# Autodesk Inventor assembly: A2017_T5_01
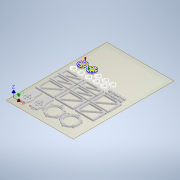
[picture p0: Inventor's stored thumbnail of the model, 180x180]
Saved by Autodesk Inventor 2020 (Build 240168000, 168)
## iProperties
Created: 2021-08-27
Part Number: A2017_T5_01
Document SubType Name: Assembly
Designer: Masato
Author: Masato
## Documents named in this file (9)
- C:\Users\marin\Documents\0113 git clone\OpenPlatform_ver3_0\cam\A2017_T5_01.iam
- C:\Users\marin\Documents\0113 git clone\OpenPlatform_ver3_0\cam\Disposable_Board.ipt
- C:\Users\marin\Documents\0113 git clone\OpenPlatform_ver3_0\LowerBody\Leg_joit\Leg_joint_yaw_frame.ipt
- C:\Users\marin\Documents\0113 git clone\OpenPlatform_ver3_0\LowerBody\Foot\Foot_root_block.ipt
- C:\Users\marin\Documents\0113 git clone\OpenPlatform_ver3_0\LowerBody\Link\FrontLink_diagonal.ipt
- C:\Users\marin\Documents\0113 git clone\OpenPlatform_ver3_0\LowerBody\Link\BackLink_diagonal.ipt
- C:\Users\marin\Documents\0113 git clone\OpenPlatform_ver3_0\UpperBody\Trunk\CrossRollerBearing\Outer_support_stand.ipt
- C:\Users\marin\Documents\0113 git clone\OpenPlatform_ver3_0\LowerBody\Knee\Knee_clamp.ipt
- C:\Users\marin\Documents\0113 git clone\OpenPlatform_ver3_0\UpperBody\Trunk\CrossRollerBearing\Inner_support_stand.ipt
## Components (27 placed, 8 different names)
1. Disposable_Board:1 — メイト:2, メイト:1, フラッシュ:1, フラッシュ:2, フラッシュ:3, 正接:1, 角度:1, 正接:4, フラッシュ:6, フラッシュ:8, 角度:4, 正接:10, 角度:5, 正接:11, 角度:6
2. Leg_joint_yaw_frame:1 — メイト:4, フラッシュ:3, 正接:1, フラッシュ:4, 正接:2, フラッシュ:5
3. Leg_joint_yaw_frame:2 — フラッシュ:4, 正接:2, フラッシュ:5, メイト:5, 正接:3, メイト:8
4. FrontLink_diagonal:4 — メイト:9, メイト:10, メイト:14, メイト:15
5. Outer_support_stand:1 — メイト:7, 角度:1, 正接:3, 正接:4
6. Outer_support_stand:3
7. FrontLink_diagonal:1 — メイト:6, フラッシュ:6, メイト:8, メイト:12
8. FrontLink_diagonal:2
9. FrontLink_diagonal:3 — メイト:10
10. BackLink_diagonal:1 — メイト:11, フラッシュ:8, メイト:12
11. BackLink_diagonal:3 — 正接:9
12. BackLink_diagonal:4 — メイト:14
13. BackLink_diagonal:5 — メイト:16, 正接:13
14. Foot_root_block:1 — メイト:13, メイト:15, メイト:16
15. Foot_root_block:2
16. Foot_root_block:3
17. Foot_root_block:4
18. Knee_clamp:3 — メイト:19, 角度:4, 正接:9, 正接:10, 正接:12
19. Knee_clamp:4
20. Knee_clamp:5
21. Knee_clamp:6
22. Knee_clamp:7
23. Inner_support_stand:1 — メイト:20, 角度:5, 正接:11, 正接:12
24. Inner_support_stand:2 — 正接:14
25. Knee_clamp:9 — メイト:21, 角度:6, 正接:13, 正接:14
26. Knee_clamp:10
27. Knee_clamp:11
## Component patterns: (2 elements, first: Outer_support_stand:1), (3 elements, first: FrontLink_diagonal:1), (4 elements, first: BackLink_diagonal:1), (4 elements, first: Foot_root_block:1), (5 elements, first: Knee_clamp:3), (2 elements, first: Inner_support_stand:1), (3 elements, first: Knee_clamp:9)
## Relationships (39: Mate 18, Tangent 10, Flush 7, Angle 4)
- メイト:2 [Mate]: Disposable_Board:1
- メイト:1 [Mate]: Disposable_Board:1
- フラッシュ:1 [Flush]: Disposable_Board:1
- フラッシュ:2 [Flush]: Disposable_Board:1
- メイト:4 [Mate]: Leg_joint_yaw_frame:1
- フラッシュ:3 [Flush] (3 mm): Disposable_Board:1 ↔ Leg_joint_yaw_frame:1
- 正接:1 [Tangent] (3 mm): Disposable_Board:1 ↔ Leg_joint_yaw_frame:1
- フラッシュ:4 [Flush]: Leg_joint_yaw_frame:1 ↔ Leg_joint_yaw_frame:2
- 正接:2 [Tangent] (3 mm): Leg_joint_yaw_frame:1 ↔ Leg_joint_yaw_frame:2
- フラッシュ:5 [Flush]: Leg_joint_yaw_frame:1 ↔ Leg_joint_yaw_frame:2
- メイト:5 [Mate]: Leg_joint_yaw_frame:2
- メイト:6 [Mate]: FrontLink_diagonal:1
- メイト:7 [Mate]: Outer_support_stand:1
- 角度:1 [Angle] (0 deg): Disposable_Board:1 ↔ Outer_support_stand:1
- 正接:3 [Tangent] (3 mm): Leg_joint_yaw_frame:2 ↔ Outer_support_stand:1
- 正接:4 [Tangent] (3 mm): Disposable_Board:1 ↔ Outer_support_stand:1
- フラッシュ:6 [Flush] (3 mm): Disposable_Board:1 ↔ FrontLink_diagonal:1
- メイト:8 [Mate] (3 mm): Leg_joint_yaw_frame:2 ↔ FrontLink_diagonal:1
- メイト:9 [Mate]: FrontLink_diagonal:4
- メイト:10 [Mate] (3 mm): FrontLink_diagonal:4 ↔ FrontLink_diagonal:3
- メイト:11 [Mate]: BackLink_diagonal:1
- フラッシュ:8 [Flush] (3 mm): Disposable_Board:1 ↔ BackLink_diagonal:1
- メイト:12 [Mate] (3 mm): FrontLink_diagonal:1 ↔ BackLink_diagonal:1
- メイト:13 [Mate]: Foot_root_block:1
- メイト:14 [Mate] (5 mm): FrontLink_diagonal:4 ↔ BackLink_diagonal:4
- メイト:15 [Mate] (3 mm): FrontLink_diagonal:4 ↔ Foot_root_block:1
- メイト:16 [Mate] (5 mm): BackLink_diagonal:5 ↔ Foot_root_block:1
- メイト:19 [Mate]: Knee_clamp:3
- 角度:4 [Angle] (0 deg): Disposable_Board:1 ↔ Knee_clamp:3
- 正接:9 [Tangent] (3 mm): BackLink_diagonal:3 ↔ Knee_clamp:3
- 正接:10 [Tangent] (3 mm): Disposable_Board:1 ↔ Knee_clamp:3
- メイト:20 [Mate]: Inner_support_stand:1
- 角度:5 [Angle] (0 deg): Disposable_Board:1 ↔ Inner_support_stand:1
- 正接:11 [Tangent] (3 mm): Disposable_Board:1 ↔ Inner_support_stand:1
- 正接:12 [Tangent] (3 mm): Knee_clamp:3 ↔ Inner_support_stand:1
- メイト:21 [Mate]: Knee_clamp:9
- 角度:6 [Angle] (0 deg): Disposable_Board:1 ↔ Knee_clamp:9
- 正接:13 [Tangent] (21 mm): BackLink_diagonal:5 ↔ Knee_clamp:9
- 正接:14 [Tangent] (6 mm): Inner_support_stand:2 ↔ Knee_clamp:9
